# Autodesk Inventor assembly: 95656
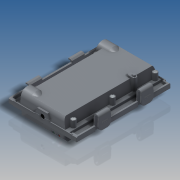
[picture p0: Inventor's stored thumbnail of the model, 180x180]
Saved by Autodesk Inventor 2016 SP2 (Build 200236200, 236)
## iProperties
Created: 2015-08-20
Part Number: 95656
Document SubType Name: Assembly
Designer: D. Kohfeld
Mass: 26.1393 g
Surface Area: 337.395 cm^2
Volume: 22.5403 cm^3
Density: 1.15967 g/cm^3
Author: D. Kohfeld
## Documents named in this file (9)
- A:\LEGO Pieces\EV3\95656.iam
- A:\LEGO Pieces\EV3\11142-LtBluishGray.ipt
- A:\LEGO Pieces\EV3\11143-LtBluishGray.ipt
- A:\LEGO Pieces\EV3\56554-ElectricAlloy.ipt
- A:\LEGO Pieces\EV3\56555-ElectricAlloy.ipt
- A:\LEGO Pieces\EV3\11177-TransGeen.ipt
- A:\LEGO Pieces\EV3\11177-TransRed.ipt
- A:\LEGO Pieces\EV3\11186-Black.ipt
- A:\LEGO Pieces\EV3\u9208.ipt
## Components (12 placed, 8 different names)
1. 11142-LtBluishGray:1 — Mate:1, Mate:2, Flush:1, Insert:3, Insert:4, Insert:5
2. 11143-LtBluishGray:1 — Mate:1, Mate:2, Flush:1, Insert:1, Insert:2, Angle:1, Angle:2, Insert:6, Insert:7, Insert:8, Insert:9, Insert:10
3. 56554-ElectricAlloy:1 — Insert:1
4. 56555-ElectricAlloy:1 — Insert:2, Angle:1
5. 11177-TransGeen:1 — Insert:3
6. 11177-TransRed:1 — Insert:4
7. 11186-Black:1 — Angle:2, Insert:5
8. u9208:1 — Insert:6
9. u9208:2 — Insert:8
10. u9208:3 — Insert:7
11. u9208:4 — Insert:9
12. u9208:5 — Insert:10
## Relationships (15: Insert 10, Mate 2, Angle 2, Flush 1)
- Mate:1: 11142-LtBluishGray:1 ↔ 11143-LtBluishGray:1
- Mate:2: 11142-LtBluishGray:1 ↔ 11143-LtBluishGray:1
- Flush:1: 11142-LtBluishGray:1 ↔ 11143-LtBluishGray:1
- Insert:1: 11143-LtBluishGray:1 ↔ 56554-ElectricAlloy:1
- Insert:2: 11143-LtBluishGray:1 ↔ 56555-ElectricAlloy:1
- Angle:1 (0 deg): 11143-LtBluishGray:1 ↔ 56555-ElectricAlloy:1
- Insert:3 (1.6 mm): 11142-LtBluishGray:1 ↔ 11177-TransGeen:1
- Insert:4 (1.6 mm): 11142-LtBluishGray:1 ↔ 11177-TransRed:1
- Angle:2 (0 deg): 11143-LtBluishGray:1 ↔ 11186-Black:1
- Insert:5: 11142-LtBluishGray:1 ↔ 11186-Black:1
- Insert:6: 11143-LtBluishGray:1 ↔ u9208:1
- Insert:7: 11143-LtBluishGray:1 ↔ u9208:3
- Insert:8: 11143-LtBluishGray:1 ↔ u9208:2
- Insert:9: 11143-LtBluishGray:1 ↔ u9208:4
- Insert:10: 11143-LtBluishGray:1 ↔ u9208:5
